# Autodesk Inventor assembly: ASY HPR 340 hopper main tube
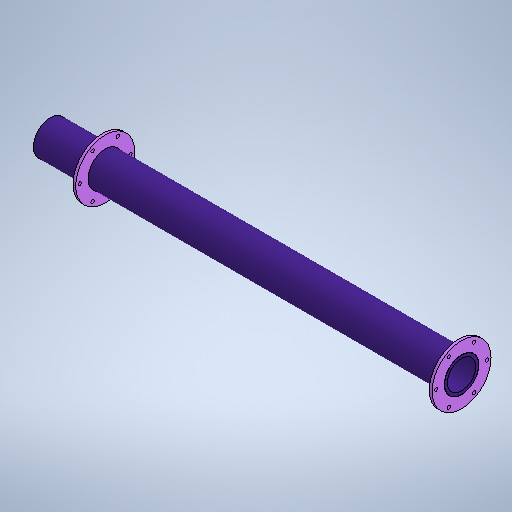
[picture p0: Inventor's stored thumbnail of the model, 512x512]
Saved by Autodesk Inventor 2025 (Build 290162010, 162A)
## iProperties
Created: 2024-12-19
Part Number: ASY HPR 340 hopper main tube
Document SubType Name: Assembly
Designer: admin
Author: admin
## Documents named in this file (3)
- C:\Users\admin\YandexDisk-badmisterfox\домашниий пк\Inventor\NDM-VOS_powder_hopper\ASY HPR 340 hopper main tube.iam
- C:\Users\admin\YandexDisk-badmisterfox\домашниий пк\Inventor\NDM-VOS_powder_hopper\NVPH-402 main tube.ipt
- C:\Users\admin\YandexDisk-badmisterfox\домашниий пк\Inventor\NDM-VOS_powder_hopper\NVPH-402 tube flange 1.ipt
## Components (3 placed, 2 different names)
1. NVPH-402 main tube:1 — Mate:1, Mate:2, Flush:1
2. NVPH-402 tube flange 1:1
3. NVPH-402 tube flange 1:2
## Relationships (5: WeldJoint 2, Mate 2, Flush 1)
- [WeldJoint] (-200 mm): NVPH-402 main tube:1 ↔ NVPH-402 tube flange 1:1
- [WeldJoint]: NVPH-402 main tube:1 ↔ NVPH-402 tube flange 1:2
- Mate:1: NVPH-402 main tube:1
- Mate:2: NVPH-402 main tube:1
- Flush:1: NVPH-402 main tube:1
